# Autodesk Inventor assembly: chassisstructure sonic shifters
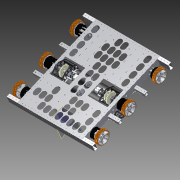
[picture p0: Inventor's stored thumbnail of the model, 180x180]
Saved by Autodesk Inventor 2014 SP1 (Build 180222100, 222)
## iProperties
Created: 2014-01-04
Part Number: chassisstructure sonic shifters
Document SubType Name: Assembly
Designer: Arpan
Mass: 5558.3 g
Surface Area: 28256.2 cm^2
Volume: 5506.27 cm^3
Density: 1.00945 g/cm^3
Author: Arpan
## Documents named in this file (18)
- C:\Users\Arpan\Documents\GitHub\2014buildCAD\chassisdrivetrain\chassis light\chassisstructure sonic shifters.iam
- C:\Users\Arpan\Documents\GitHub\2014buildCAD\chassisdrivetrain\chassis light\chassis side rail.ipt
- C:\Users\Arpan\Documents\GitHub\2014buildCAD\chassisdrivetrain\gearbot\3cimgearbox.iam
- C:\Users\Arpan\Documents\GitHub\2014buildCAD\chassisdrivetrain\chassis light\COTS items\center wheel assembly.iam
- C:\Users\Arpan\Documents\GitHub\2014buildCAD\chassisdrivetrain\chassis light\COTS items\.5 inch bearing pretend its hex.ipt
- C:\Users\Arpan\Documents\GitHub\2014buildCAD\chassisdrivetrain\chassis light\4.5 hex shaft.ipt
- C:\Users\Arpan\Documents\GitHub\2014buildCAD\chassisdrivetrain\chassis light\COTS items\front wheels.iam
- C:\Users\Arpan\Documents\GitHub\2014buildCAD\chassisdrivetrain\chassis light\COTS items\back wheels.iam
- C:\Users\Arpan\Documents\GitHub\2014buildCAD\chassisdrivetrain\chassis light\COTS items\DBK_42ToothPulley V2.iam
- C:\Users\Arpan\Documents\GitHub\2014buildCAD\chassisdrivetrain\chassis light\3d printed items\back wheel spacer.ipt
- C:\Users\Arpan\Documents\GitHub\2014buildCAD\chassisdrivetrain\chassis light\PVC pipe spacer.ipt
- C:\Users\Arpan\Documents\GitHub\2014buildCAD\chassisdrivetrain\chassis light\PVC pipe spacer center wheels.ipt
- C:\Users\Arpan\Documents\GitHub\2014buildCAD\chassisdrivetrain\chassis light\baseplate.ipt
- C:\Users\Arpan\Documents\GitHub\2014buildCAD\chassisdrivetrain\chassis light\battery mount.ipt
- C:\Users\Arpan\Documents\GitHub\2014buildCAD\chassisdrivetrain\chassis light\side bumper mount.ipt
- C:\Users\Arpan\Documents\GitHub\2014buildCAD\chassisdrivetrain\chassis light\COTS items\217-3547-STEP.ipt
- C:\Users\Arpan\Documents\GitHub\2014buildCAD\chassisdrivetrain\chassis light\front back rail vexpro.ipt
- C:\Users\Arpan\Documents\GitHub\2014buildCAD\chassisdrivetrain\chassis light\back rail vexpro.ipt
## Components (44 placed, 17 different names)
1. chassis side rail:1 — Mate:6, Mate:7, Mate:14, Mate:15, Mate:16, Mate:17, Mate:18, Mate:19, Mate:20, Mate:29, Mate:56, Mate:58, Mate:62, Mate:67, Mate:72, Flush:28, Mate:73, Flush:29, Mate:75, Flush:31, Flush:33, Mate:83, Flush:41, Flush:43, Flush:44, Mate:92
2. chassis side rail:2 — Mate:8, Mate:9, Mate:21, Mate:22, Mate:23, Mate:24, Mate:25, Mate:26, Mate:27, Mate:28, Angle:3, Mate:54, Mate:60, Mate:64, Flush:25, Mate:70, Mate:71, Flush:26, Flush:27, Flush:36, Mate:78, Flush:37, Mate:82, Flush:39, Mate:86, Flush:43
3. 3cimgearbox:1 [sub-assembly] — Mate:6, Mate:7, Angle:2, Flush:7, Mate:12, Mate:13, Mate:61
4. 3cimgearbox:2 [sub-assembly] — Mate:8, Mate:9, Angle:2, Flush:6, Mate:10, Mate:11, Mate:63
5. center wheel assembly:1 [sub-assembly] — Flush:6, Mate:10, Mate:11, Flush:17, Flush:18, Flush:22
6. center wheel assembly:2 [sub-assembly] — Flush:7, Mate:12, Mate:13, Flush:21, Flush:23
7. .5 inch bearing pretend its hex:1 — Mate:16, Mate:17
8. .5 inch bearing pretend its hex:2 — Mate:14, Mate:15, Mate:30
9. .5 inch bearing pretend its hex:3 — Mate:19, Mate:29
10. .5 inch bearing pretend its hex:4 — Mate:18, Mate:20, Mate:31
11. .5 inch bearing pretend its hex:5 — Mate:21, Mate:24, Mate:33
12. .5 inch bearing pretend its hex:6 — Mate:22, Mate:23
13. .5 inch bearing pretend its hex:7 — Mate:25, Mate:26, Mate:32
14. .5 inch bearing pretend its hex:8 — Mate:27, Mate:28
15. 4.5 hex shaft:1 — Mate:30, Flush:9, Flush:13, Mate:36, Mate:37, Mate:55
16. 4.5 hex shaft:2 — Mate:31, Flush:9, Flush:15, Mate:40, Mate:41, Mate:57
17. 4.5 hex shaft:3 — Mate:32, Flush:11, Mate:34, Mate:35, Angle:3, Flush:19, Mate:59
18. 4.5 hex shaft:4 — Flush:11, Mate:33, Mate:38, Mate:39, Flush:20, Mate:53
19. front wheels:1 [sub-assembly] — Mate:34, Mate:35, Flush:17, Flush:19
20. front wheels:2 [sub-assembly] — Flush:13, Mate:36, Mate:37, Flush:21
21. back wheels:1 [sub-assembly] — Flush:15, Mate:40, Mate:41, Mate:42, Mate:43, Mate:44, Mate:48, Mate:49
22. back wheels:2 [sub-assembly] — Mate:38, Mate:39, Mate:45, Mate:46, Flush:18, Flush:20, Mate:51, Mate:52
23. DBK_42ToothPulley V2:1 [sub-assembly] — Mate:42, Mate:43, Mate:44, Flush:23, Mate:47
24. DBK_42ToothPulley V2:2 [sub-assembly] — Mate:45, Mate:46, Flush:22, Mate:50
25. back wheel spacer:1 — Mate:47, Mate:48, Mate:49
26. back wheel spacer:2 — Mate:50, Mate:51, Mate:52
27. PVC pipe spacer:1 — Mate:55, Mate:56
28. PVC pipe spacer:2 — Mate:57, Mate:58
29. PVC pipe spacer:3 — Mate:53, Mate:54
30. PVC pipe spacer:4 — Mate:59, Mate:60
31. PVC pipe spacer center wheels:1 — Mate:61, Mate:62
32. PVC pipe spacer center wheels:2 — Mate:63, Mate:64
33. baseplate:1 — Flush:25, Mate:79, Mate:80, Mate:81, Flush:40, Mate:86, Mate:91
34. battery mount:1 — Mate:67, Mate:79, Mate:93
35. side bumper mount:1 — Mate:70, Flush:27, Flush:30, Mate:77, Flush:35, Mate:90
36. side bumper mount:2 — Mate:71, Flush:26, Flush:38, Flush:45, Mate:90, Flush:46
37. side bumper mount:3 — Mate:72, Flush:28, Flush:30, Flush:32
38. side bumper mount:4 — Mate:73, Flush:29, Mate:76, Flush:34, Flush:45
39. 217-3547-STEP:1 — Mate:75, Flush:31, Flush:32
40. 217-3547-STEP:2 — Mate:76, Flush:33, Flush:34
41. 217-3547-STEP:3 — Mate:77, Flush:35, Flush:36
42. 217-3547-STEP:4 — Mate:78, Flush:37, Flush:38
43. front back rail vexpro:1 — Mate:80, Mate:81, Mate:82, Flush:39, Mate:83, Flush:40, Flush:41, Flush:44, Flush:46, Flush:47
44. back rail vexpro:1 — Mate:91, Flush:47, Mate:92, Mate:93
## Relationships (115: Mate 78, Flush 35, Angle 2)
- Mate:6: chassis side rail:1 ↔ 3cimgearbox:1
- Mate:7: chassis side rail:1 ↔ 3cimgearbox:1
- Mate:8: chassis side rail:2 ↔ 3cimgearbox:2
- Mate:9: chassis side rail:2 ↔ 3cimgearbox:2
- Angle:2 (0 deg): 3cimgearbox:1 ↔ 3cimgearbox:2
- Flush:6: 3cimgearbox:2 ↔ center wheel assembly:1
- Mate:10: 3cimgearbox:2 ↔ center wheel assembly:1
- Mate:11: 3cimgearbox:2 ↔ center wheel assembly:1
- Flush:7: 3cimgearbox:1 ↔ center wheel assembly:2
- Mate:12: 3cimgearbox:1 ↔ center wheel assembly:2
- Mate:13: 3cimgearbox:1 ↔ center wheel assembly:2
- Mate:14: chassis side rail:1 ↔ .5 inch bearing pretend its hex:2
- Mate:15: chassis side rail:1 ↔ .5 inch bearing pretend its hex:2
- Mate:16: chassis side rail:1 ↔ .5 inch bearing pretend its hex:1
- Mate:17: chassis side rail:1 ↔ .5 inch bearing pretend its hex:1
- Mate:18: chassis side rail:1 ↔ .5 inch bearing pretend its hex:4
- Mate:19: chassis side rail:1 ↔ .5 inch bearing pretend its hex:3
- Mate:20: chassis side rail:1 ↔ .5 inch bearing pretend its hex:4
- Mate:21: chassis side rail:2 ↔ .5 inch bearing pretend its hex:5
- Mate:22: chassis side rail:2 ↔ .5 inch bearing pretend its hex:6
- Mate:23: chassis side rail:2 ↔ .5 inch bearing pretend its hex:6
- Mate:24: chassis side rail:2 ↔ .5 inch bearing pretend its hex:5
- Mate:25: chassis side rail:2 ↔ .5 inch bearing pretend its hex:7
- Mate:26: chassis side rail:2 ↔ .5 inch bearing pretend its hex:7
- Mate:27: chassis side rail:2 ↔ .5 inch bearing pretend its hex:8
- Mate:28: chassis side rail:2 ↔ .5 inch bearing pretend its hex:8
- Mate:29: chassis side rail:1 ↔ .5 inch bearing pretend its hex:3
- Mate:30: .5 inch bearing pretend its hex:2 ↔ 4.5 hex shaft:1
- Mate:31: .5 inch bearing pretend its hex:4 ↔ 4.5 hex shaft:2
- Flush:9: 4.5 hex shaft:1 ↔ 4.5 hex shaft:2
- Mate:32: .5 inch bearing pretend its hex:7 ↔ 4.5 hex shaft:3
- Flush:11: 4.5 hex shaft:3 ↔ 4.5 hex shaft:4
- Mate:33: .5 inch bearing pretend its hex:5 ↔ 4.5 hex shaft:4
- Mate:34: 4.5 hex shaft:3 ↔ front wheels:1
- Mate:35: 4.5 hex shaft:3 ↔ front wheels:1
- Flush:13: 4.5 hex shaft:1 ↔ front wheels:2
- Mate:36: 4.5 hex shaft:1 ↔ front wheels:2
- Mate:37: 4.5 hex shaft:1 ↔ front wheels:2
- Mate:38: 4.5 hex shaft:4 ↔ back wheels:2
- Mate:39: 4.5 hex shaft:4 ↔ back wheels:2
- Flush:15: 4.5 hex shaft:2 ↔ back wheels:1
- Mate:40: 4.5 hex shaft:2 ↔ back wheels:1
- Mate:41: 4.5 hex shaft:2 ↔ back wheels:1
- Mate:42: back wheels:1 ↔ DBK_42ToothPulley V2:1
- Mate:43: back wheels:1 ↔ DBK_42ToothPulley V2:1
- Mate:44: back wheels:1 ↔ DBK_42ToothPulley V2:1
- Mate:45: back wheels:2 ↔ DBK_42ToothPulley V2:2
- Mate:46: back wheels:2 ↔ DBK_42ToothPulley V2:2
- Flush:17: center wheel assembly:1 ↔ front wheels:1
- Flush:18: center wheel assembly:1 ↔ back wheels:2
- Angle:3 (0 deg): chassis side rail:2 ↔ 4.5 hex shaft:3
- Flush:19: 4.5 hex shaft:3 ↔ front wheels:1
- Flush:20: 4.5 hex shaft:4 ↔ back wheels:2
- Flush:21: center wheel assembly:2 ↔ front wheels:2
- Flush:22: center wheel assembly:1 ↔ DBK_42ToothPulley V2:2
- Flush:23: center wheel assembly:2 ↔ DBK_42ToothPulley V2:1
- Mate:47: DBK_42ToothPulley V2:1 ↔ back wheel spacer:1
- Mate:48: back wheels:1 ↔ back wheel spacer:1
- Mate:49: back wheels:1 ↔ back wheel spacer:1
- Mate:50: DBK_42ToothPulley V2:2 ↔ back wheel spacer:2
- Mate:51: back wheels:2 ↔ back wheel spacer:2
- Mate:52: back wheels:2 ↔ back wheel spacer:2
- Mate:53: 4.5 hex shaft:4 ↔ PVC pipe spacer:3
- Mate:54: chassis side rail:2 ↔ PVC pipe spacer:3
- Mate:55: 4.5 hex shaft:1 ↔ PVC pipe spacer:1
- Mate:56: chassis side rail:1 ↔ PVC pipe spacer:1
- Mate:57: 4.5 hex shaft:2 ↔ PVC pipe spacer:2
- Mate:58: chassis side rail:1 ↔ PVC pipe spacer:2
- Mate:59: 4.5 hex shaft:3 ↔ PVC pipe spacer:4
- Mate:60: chassis side rail:2 ↔ PVC pipe spacer:4
- Mate:61: 3cimgearbox:1 ↔ PVC pipe spacer center wheels:1
- Mate:62: chassis side rail:1 ↔ PVC pipe spacer center wheels:1
- Mate:63: 3cimgearbox:2 ↔ PVC pipe spacer center wheels:2
- Mate:64: chassis side rail:2 ↔ PVC pipe spacer center wheels:2
- Flush:25: chassis side rail:2 ↔ baseplate:1
- Mate:67 (49.53 mm): chassis side rail:1 ↔ battery mount:1
- Mate:70: chassis side rail:2 ↔ side bumper mount:1
- Mate:71: chassis side rail:2 ↔ side bumper mount:2
- Flush:26: chassis side rail:2 ↔ side bumper mount:2
- Flush:27: chassis side rail:2 ↔ side bumper mount:1
- Mate:72: chassis side rail:1 ↔ side bumper mount:3
- Flush:28: chassis side rail:1 ↔ side bumper mount:3
- Mate:73: chassis side rail:1 ↔ side bumper mount:4
- Flush:29: chassis side rail:1 ↔ side bumper mount:4
- Flush:30: side bumper mount:1 ↔ side bumper mount:3
- Mate:75: chassis side rail:1 ↔ 217-3547-STEP:1
- Flush:31: chassis side rail:1 ↔ 217-3547-STEP:1
- Flush:32: side bumper mount:3 ↔ 217-3547-STEP:1
- Mate:76: side bumper mount:4 ↔ 217-3547-STEP:2
- Flush:33: chassis side rail:1 ↔ 217-3547-STEP:2
- Flush:34: side bumper mount:4 ↔ 217-3547-STEP:2
- Mate:77: side bumper mount:1 ↔ 217-3547-STEP:3
- Flush:35: side bumper mount:1 ↔ 217-3547-STEP:3
- Flush:36: chassis side rail:2 ↔ 217-3547-STEP:3
- Mate:78: chassis side rail:2 ↔ 217-3547-STEP:4
- Flush:37: chassis side rail:2 ↔ 217-3547-STEP:4
- Flush:38: side bumper mount:2 ↔ 217-3547-STEP:4
- Mate:79: baseplate:1 ↔ battery mount:1
- Mate:80: baseplate:1 ↔ front back rail vexpro:1
- Mate:81: baseplate:1 ↔ front back rail vexpro:1
- Mate:82: chassis side rail:2 ↔ front back rail vexpro:1
- Flush:39 (86.36 mm): chassis side rail:2 ↔ front back rail vexpro:1
- Mate:83: chassis side rail:1 ↔ front back rail vexpro:1
- Flush:40: baseplate:1 ↔ front back rail vexpro:1
- Flush:41: chassis side rail:1 ↔ front back rail vexpro:1
- Mate:86: chassis side rail:2 ↔ baseplate:1
- Flush:43: chassis side rail:1 ↔ chassis side rail:2
- Flush:44 (86.36 mm): chassis side rail:1 ↔ front back rail vexpro:1
- Flush:45: side bumper mount:2 ↔ side bumper mount:4
- Mate:90 (203.2 mm): side bumper mount:1 ↔ side bumper mount:2
- Flush:46 (-444.5 mm): side bumper mount:2 ↔ front back rail vexpro:1
- Mate:91: baseplate:1 ↔ back rail vexpro:1
- Flush:47: front back rail vexpro:1 ↔ back rail vexpro:1
- Mate:92: chassis side rail:1 ↔ back rail vexpro:1
- Mate:93: battery mount:1 ↔ back rail vexpro:1
